# Autodesk Inventor assembly: 202.001.01_Vereinzelung_Gesamtbaugruppe
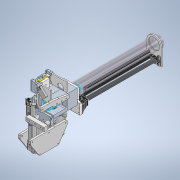
[picture p0: Inventor's stored thumbnail of the model, 180x180]
Saved by Autodesk Inventor 2021 (Build 250183000, 183)
## iProperties
Created: 2021-11-14
Part Number: 202.001.01_Vereinzelung_Gesamtbaugruppe
Document SubType Name: Assembly
Designer: Oliver Ungerer
Sending System: Creo  TM  4.0
KODE_ZEICHNUNGSNUMMER: TFVEM_100M
BENENNUNG: Vereinzelungsmechanismus
BEARBEITER_NAME: Ungerer O.
MASSE: 6.946813
PDMREV: 0.0+
PDMRL: Entwicklung
PROI_REVISION: 0
PROI_VERSION: 0+
PROI_RELEASE: Entwicklung
PTC_MODIFIED: True
PROI_CREATED_BY: Kantioler_adm
PROI_CREATED_ON: 07.03.2008 12:11:19
PROI_LOCATION: Root-Ordner/Pro_stds/Start_Files
MATERIALART: -
EINHEIT: ST
HERSTELLER_PREIS: 0.0
PRUEFER_NAME: Uo
PTC_ORGANIZATION_ID: Durst
PTC_WM_REVISION: 0
PTC_WM_ITERATION: 0
PTC_WM_VERSION: 0.0
PTC_WM_LIFECYCLE_STATE: Entwicklung
PTC_WM_LIFECYCLE: 02 Durst
PTC_WM_CREATED_BY: Oliver Ungerer (oungerer: Durst)
PTC_WM_CREATED_ON: 01.08.21
PTC_WM_MODIFIED_BY: Oliver Ungerer (oungerer: Durst)
PTC_WM_MODIFIED_ON: 01.08.21
AEND_INDEX: 0
VERSION: 0
STATUS: 0.0
Author: Oliver Ungerer
## Documents named in this file (22)
- C:\Users\Sebastian Seewald\Documents\Inventor\Konstruktion_Studium\Lernfabrik\106_Vereinzelungseinheit\202.001.01_Vereinzelung_Gesamtbaugruppe.iam
- 206.001.01_Vereinzelung_Gesamtbaugruppe.iam
- C:\Users\Sebastian Seewald\Documents\Inventor\Konstruktion_Studium\Lernfabrik\106_Vereinzelungseinheit\TFVEM_1000.ipt
- C:\Users\Sebastian Seewald\Documents\Inventor\Konstruktion_Studium\Lernfabrik\106_Vereinzelungseinheit\TFVEM_1001.ipt
- C:\Users\Sebastian Seewald\Documents\Inventor\Konstruktion_Studium\Lernfabrik\106_Vereinzelungseinheit\TFVEM_1002.ipt
- C:\Users\Sebastian Seewald\Documents\Inventor\Konstruktion_Studium\Lernfabrik\106_Vereinzelungseinheit\TFVEM_1003.ipt
- C:\Users\Sebastian Seewald\Documents\Inventor\Konstruktion_Studium\Lernfabrik\106_Vereinzelungseinheit\0001_FLASCHE.ipt
- C:\Users\Sebastian Seewald\Documents\Inventor\Konstruktion_Studium\Lernfabrik\106_Vereinzelungseinheit\TFVEM_1007.ipt
- C:\Users\Sebastian Seewald\Documents\Inventor\Konstruktion_Studium\Lernfabrik\106_Vereinzelungseinheit\TFVEM_1010.ipt
- C:\Users\Sebastian Seewald\Documents\Inventor\Konstruktion_Studium\Lernfabrik\106_Vereinzelungseinheit\_BALLUFF_BIS_M-305-ANTENNE.ipt
- C:\Users\Sebastian Seewald\Documents\Inventor\Konstruktion_Studium\Lernfabrik\106_Vereinzelungseinheit\TFVEM_1011.ipt
- C:\Users\Sebastian Seewald\Documents\Inventor\Konstruktion_Studium\Lernfabrik\106_Vereinzelungseinheit\BALLUFF_BCS_M18BBN1-PSC80D-EP02.ipt
- C:\Users\Sebastian Seewald\Documents\Inventor\Konstruktion_Studium\Lernfabrik\106_Vereinzelungseinheit\TFVEM_1020.ipt
- C:\Users\Sebastian Seewald\Documents\Inventor\Konstruktion_Studium\Lernfabrik\106_Vereinzelungseinheit\TFVEM_1021.ipt
- C:\Users\Sebastian Seewald\Documents\Inventor\Konstruktion_Studium\Lernfabrik\106_Vereinzelungseinheit\TFVEM_1022.ipt
- C:\Users\Sebastian Seewald\Documents\Inventor\Konstruktion_Studium\Lernfabrik\106_Vereinzelungseinheit\TFVEM_1023.ipt
- C:\Users\Sebastian Seewald\Documents\Inventor\Konstruktion_Studium\Lernfabrik\106_Vereinzelungseinheit\TFVEM_1024.ipt
- C:\Users\Sebastian Seewald\Documents\Inventor\Konstruktion_Studium\Lernfabrik\106_Vereinzelungseinheit\TFVEM_1025.ipt
- C:\Users\Sebastian Seewald\Documents\Inventor\Konstruktion_Studium\Lernfabrik\106_Vereinzelungseinheit\102.003.01_Anbindung_Vereinzelung.ipt
- C:\Users\Sebastian Seewald\Documents\Inventor\Konstruktion_Studium\Lernfabrik\106_Vereinzelungseinheit\202.002.01_Schieberbetaetigung.iam
- C:\Users\Sebastian Seewald\Documents\Inventor\Konstruktion_Studium\Lernfabrik\106_Vereinzelungseinheit\102.001.01_Anbindung_Vereinzelung.ipt
- C:\Users\Sebastian Seewald\Documents\Inventor\Konstruktion_Studium\Lernfabrik\106_Vereinzelungseinheit\102.002.01_Justage_Vereinzelung.ipt
## Components (25 placed, 20 different names)
1. 106.001.01_Aufnahmeblock_links — Passend:15, Passend:16, Passend:17, Passend:18, Passend:21, Passend:25, Passend:27, Passend:43, Passend:47, Passend:48, Passend:49
2. 106.002.01_Fuehrungsblock_rechts — Passend:13, Fluchtend:1, Passend:14, Fluchtend:2, Passend:15, Passend:16, Passend:17, Fluchtend:3, Passend:26, Fluchtend:4, Fluchtend:5, Passend:44, Passend:45, Fluchtend:12
3. 206.001.01_Schieberbetaetigung [sub-assembly] — Passend:2, Passend:3, Passend:4, Passend:52, Passend:53, Passend:54
4. 106.003.01_Aufnahmeblock_oben — Passend:14, Fluchtend:2, Passend:21, Passend:22, Passend:23, Passend:24, Passend:30, Passend:31, Passend:32
5. 106.004.01_Aufnahme_Rahmen — Passend:6, Passend:7, Passend:8, Passend:10, Passend:12, Passend:43, Passend:44, Passend:45
6. 506.001.01_Laborflaschen — Passend:18, Fluchtend:3, Passend:19, Passend:20
7. 506.001.01_Laborflaschen:1 — Passend:19, Passend:20
8. 106.005.01_Befuellungsrohr — Passend:40, Passend:41, Passend:42
9. 106.006.01_Schieberaufnahme — Passend:2, Passend:3, Passend:4, Passend:47, Passend:48, Passend:49
10. 506.002.01_BALLUFF_BIS_M-305-ANTENNE — Passend:52, Passend:53, Passend:54
11. 106.007.01_Aufnahme_Sensor — Passend:22, Passend:23, Passend:24, Passend:28
12. 106.007.01_Aufnahme_Sensor:1 — Passend:25, Passend:26, Passend:27, Passend:29
13. 506.003.01_BALLUFF_BCS_M18BBN1-PSC80D-EP02 — Passend:28, Fluchtend:4
14. 506.003.01_BALLUFF_BCS_M18BBN1-PSC80D-EP02:1 — Passend:29, Fluchtend:5
15. 506.003.01_BALLUFF_BCS_M18BBN1-PSC80D-EP02:3 — Passend:46, Fluchtend:10
16. 106.008.01_Aufnahme_Buerste — Passend:30, Passend:31, Passend:32, Passend:33, Fluchtend:6, Fluchtend:7, Fluchtend:8, Fluchtend:9, Passend:34, Passend:40
17. 106.009.01_Halterung_Sensor_oben — Passend:33, Fluchtend:6, Fluchtend:7, Passend:41, Passend:46, Fluchtend:10
18. 106.010.01_Buerstenbremse — Passend:35, Passend:36, Winkel:1, Passend:37, Passend:38, Winkel:2
19. 106.011.01_Aufnahme_Buerstenbremse_unten — Fluchtend:8, Fluchtend:9, Passend:34, Passend:35, Passend:36, Winkel:1
20. 106.012.01_Aufnahme_Buerstenbremse_oben — Passend:37, Passend:38, Winkel:2, Passend:39, Winkel:3
21. 106.013.01_Halterung_Burstenbremse_oben — Passend:39, Passend:42, Winkel:3
22. 106.014.01_Anbindung_Vereinzelung:1 — Passend:6, Passend:7, Passend:8, Passend:9, Passend:11
23. 106.015.01_Justage_Vereinzelung:2 — Passend:9, Passend:10
24. 106.015.01_Justage_Vereinzelung:1 — Passend:11, Passend:12
25. 106.016.01_Anbindung_Vereinzelung:4 — Passend:13, Fluchtend:1, Fluchtend:12
## Relationships (64: Mate 50, Flush 11, Angle 3)
- Passend:2 [Mate]: 206.001.01_Schieberbetaetigung ↔ 106.006.01_Schieberaufnahme
- Passend:3 [Mate]: 206.001.01_Schieberbetaetigung ↔ 106.006.01_Schieberaufnahme
- Passend:4 [Mate]: 206.001.01_Schieberbetaetigung ↔ 106.006.01_Schieberaufnahme
- Passend:6 [Mate]: 106.004.01_Aufnahme_Rahmen ↔ 106.014.01_Anbindung_Vereinzelung:1
- Passend:7 [Mate]: 106.004.01_Aufnahme_Rahmen ↔ 106.014.01_Anbindung_Vereinzelung:1
- Passend:8 [Mate] (25 mm): 106.004.01_Aufnahme_Rahmen ↔ 106.014.01_Anbindung_Vereinzelung:1
- Passend:9 [Mate]: 106.014.01_Anbindung_Vereinzelung:1 ↔ 106.015.01_Justage_Vereinzelung:2
- Passend:10 [Mate]: 106.004.01_Aufnahme_Rahmen ↔ 106.015.01_Justage_Vereinzelung:2
- Passend:11 [Mate]: 106.014.01_Anbindung_Vereinzelung:1 ↔ 106.015.01_Justage_Vereinzelung:1
- Passend:12 [Mate]: 106.004.01_Aufnahme_Rahmen ↔ 106.015.01_Justage_Vereinzelung:1
- Passend:13 [Mate]: 106.002.01_Fuehrungsblock_rechts ↔ 106.016.01_Anbindung_Vereinzelung:4
- Fluchtend:1 [Flush]: 106.002.01_Fuehrungsblock_rechts ↔ 106.016.01_Anbindung_Vereinzelung:4
- Passend:14 [Mate]: 106.002.01_Fuehrungsblock_rechts ↔ 106.003.01_Aufnahmeblock_oben
- Fluchtend:2 [Flush]: 106.002.01_Fuehrungsblock_rechts ↔ 106.003.01_Aufnahmeblock_oben
- Passend:15 [Mate]: 106.001.01_Aufnahmeblock_links ↔ 106.002.01_Fuehrungsblock_rechts
- Passend:16 [Mate]: 106.001.01_Aufnahmeblock_links ↔ 106.002.01_Fuehrungsblock_rechts
- Passend:17 [Mate]: 106.001.01_Aufnahmeblock_links ↔ 106.002.01_Fuehrungsblock_rechts
- Passend:18 [Mate]: 106.001.01_Aufnahmeblock_links ↔ 506.001.01_Laborflaschen
- Fluchtend:3 [Flush]: 106.002.01_Fuehrungsblock_rechts ↔ 506.001.01_Laborflaschen
- Passend:19 [Mate]: 506.001.01_Laborflaschen ↔ 506.001.01_Laborflaschen:1
- Passend:20 [Mate]: 506.001.01_Laborflaschen ↔ 506.001.01_Laborflaschen:1
- Passend:21 [Mate]: 106.001.01_Aufnahmeblock_links ↔ 106.003.01_Aufnahmeblock_oben
- Passend:22 [Mate]: 106.003.01_Aufnahmeblock_oben ↔ 106.007.01_Aufnahme_Sensor
- Passend:23 [Mate]: 106.003.01_Aufnahmeblock_oben ↔ 106.007.01_Aufnahme_Sensor
- Passend:24 [Mate]: 106.003.01_Aufnahmeblock_oben ↔ 106.007.01_Aufnahme_Sensor
- Passend:25 [Mate]: 106.001.01_Aufnahmeblock_links ↔ 106.007.01_Aufnahme_Sensor:1
- Passend:26 [Mate]: 106.002.01_Fuehrungsblock_rechts ↔ 106.007.01_Aufnahme_Sensor:1
- Passend:27 [Mate]: 106.001.01_Aufnahmeblock_links ↔ 106.007.01_Aufnahme_Sensor:1
- Passend:28 [Mate]: 106.007.01_Aufnahme_Sensor ↔ 506.003.01_BALLUFF_BCS_M18BBN1-PSC80D-EP02
- Fluchtend:4 [Flush]: 106.002.01_Fuehrungsblock_rechts ↔ 506.003.01_BALLUFF_BCS_M18BBN1-PSC80D-EP02
- Passend:29 [Mate]: 106.007.01_Aufnahme_Sensor:1 ↔ 506.003.01_BALLUFF_BCS_M18BBN1-PSC80D-EP02:1
- Fluchtend:5 [Flush]: 106.002.01_Fuehrungsblock_rechts ↔ 506.003.01_BALLUFF_BCS_M18BBN1-PSC80D-EP02:1
- Passend:30 [Mate]: 106.003.01_Aufnahmeblock_oben ↔ 106.008.01_Aufnahme_Buerste
- Passend:31 [Mate]: 106.003.01_Aufnahmeblock_oben ↔ 106.008.01_Aufnahme_Buerste
- Passend:32 [Mate]: 106.003.01_Aufnahmeblock_oben ↔ 106.008.01_Aufnahme_Buerste
- Passend:33 [Mate]: 106.008.01_Aufnahme_Buerste ↔ 106.009.01_Halterung_Sensor_oben
- Fluchtend:6 [Flush]: 106.008.01_Aufnahme_Buerste ↔ 106.009.01_Halterung_Sensor_oben
- Fluchtend:7 [Flush]: 106.008.01_Aufnahme_Buerste ↔ 106.009.01_Halterung_Sensor_oben
- Fluchtend:8 [Flush]: 106.008.01_Aufnahme_Buerste ↔ 106.011.01_Aufnahme_Buerstenbremse_unten
- Fluchtend:9 [Flush]: 106.008.01_Aufnahme_Buerste ↔ 106.011.01_Aufnahme_Buerstenbremse_unten
- Passend:34 [Mate]: 106.008.01_Aufnahme_Buerste ↔ 106.011.01_Aufnahme_Buerstenbremse_unten
- Passend:35 [Mate]: 106.010.01_Buerstenbremse ↔ 106.011.01_Aufnahme_Buerstenbremse_unten
- Passend:36 [Mate]: 106.010.01_Buerstenbremse ↔ 106.011.01_Aufnahme_Buerstenbremse_unten
- Winkel:1 [Angle] (180 deg): 106.010.01_Buerstenbremse ↔ 106.011.01_Aufnahme_Buerstenbremse_unten
- Passend:37 [Mate]: 106.010.01_Buerstenbremse ↔ 106.012.01_Aufnahme_Buerstenbremse_oben
- Passend:38 [Mate]: 106.010.01_Buerstenbremse ↔ 106.012.01_Aufnahme_Buerstenbremse_oben
- Winkel:2 [Angle] (180 deg): 106.010.01_Buerstenbremse ↔ 106.012.01_Aufnahme_Buerstenbremse_oben
- Passend:39 [Mate]: 106.012.01_Aufnahme_Buerstenbremse_oben ↔ 106.013.01_Halterung_Burstenbremse_oben
- Passend:40 [Mate]: 106.005.01_Befuellungsrohr ↔ 106.008.01_Aufnahme_Buerste
- Passend:41 [Mate]: 106.005.01_Befuellungsrohr ↔ 106.009.01_Halterung_Sensor_oben
- Passend:42 [Mate]: 106.005.01_Befuellungsrohr ↔ 106.013.01_Halterung_Burstenbremse_oben
- Winkel:3 [Angle] (0 deg): 106.012.01_Aufnahme_Buerstenbremse_oben ↔ 106.013.01_Halterung_Burstenbremse_oben
- Passend:43 [Mate]: 106.001.01_Aufnahmeblock_links ↔ 106.004.01_Aufnahme_Rahmen
- Passend:44 [Mate]: 106.002.01_Fuehrungsblock_rechts ↔ 106.004.01_Aufnahme_Rahmen
- Passend:45 [Mate]: 106.002.01_Fuehrungsblock_rechts ↔ 106.004.01_Aufnahme_Rahmen
- Passend:46 [Mate]: 506.003.01_BALLUFF_BCS_M18BBN1-PSC80D-EP02:3 ↔ 106.009.01_Halterung_Sensor_oben
- Fluchtend:10 [Flush] (10 mm): 506.003.01_BALLUFF_BCS_M18BBN1-PSC80D-EP02:3 ↔ 106.009.01_Halterung_Sensor_oben
- Passend:47 [Mate]: 106.001.01_Aufnahmeblock_links ↔ 106.006.01_Schieberaufnahme
- Passend:48 [Mate]: 106.001.01_Aufnahmeblock_links ↔ 106.006.01_Schieberaufnahme
- Passend:49 [Mate]: 106.001.01_Aufnahmeblock_links ↔ 106.006.01_Schieberaufnahme
- Passend:52 [Mate]: 206.001.01_Schieberbetaetigung ↔ 506.002.01_BALLUFF_BIS_M-305-ANTENNE
- Passend:53 [Mate]: 206.001.01_Schieberbetaetigung ↔ 506.002.01_BALLUFF_BIS_M-305-ANTENNE
- Passend:54 [Mate]: 206.001.01_Schieberbetaetigung ↔ 506.002.01_BALLUFF_BIS_M-305-ANTENNE
- Fluchtend:12 [Flush]: 106.002.01_Fuehrungsblock_rechts ↔ 106.016.01_Anbindung_Vereinzelung:4
